# Autodesk Inventor assembly: 3 Postion Pneumatic Cylinder (9-16 in Bore, .25 in,2 in stroke)
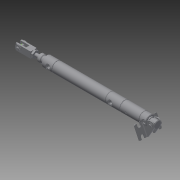
[picture p0: Inventor's stored thumbnail of the model, 180x180]
Saved by Autodesk Inventor 2014 (Build 180170000, 170)
## iProperties
Created: 2014-01-17
Part Number: 3 Postion Pneumatic Cylinder (9-16 in Bore, .25 in,2 in stroke)
Document SubType Name: Assembly
Designer: Michael
Mass: 25.114 g
Surface Area: 262.97 cm^2
Volume: 25.114 cm^3
Density: 1 g/cm^3
Title: //expscmdclustefs.cadenas.external/client_exchange/iodir/jobs/output/wkb68069816_no0/STEP/020_25_2-DXP_D-850__D-12321-A__2_03.stp
Description: STEP AP203
Sending System: PARTsolutions
Preprocessor: PSStep 15.0.47
Author: Michael
## Documents named in this file (20)
- C:\Users\Michael\Documents\GitHub\2014buildCAD\New Collector\3 Postion Pneumatic Cylinder (9-16 in Bore, .25 in,2 in stroke).iam
- C:\Users\Michael\Documents\GitHub\2014buildCAD\Imported Components\020_25_2-DXP_D-850__D-12321-A__2_03\HI_020.25_2-DXP(D-850)(D-12321-A)0_dummy.ipt
- C:\Users\Michael\Documents\GitHub\2014buildCAD\Imported Components\020_25_2-DXP_D-850__D-12321-A__2_03\HI_D-68355-XP--0.ipt
- C:\Users\Michael\Documents\GitHub\2014buildCAD\Imported Components\020_25_2-DXP_D-850__D-12321-A__2_03\HI_D-75938XP-1.188.ipt
- C:\Users\Michael\Documents\GitHub\2014buildCAD\Imported Components\020_25_2-DXP_D-850__D-12321-A__2_03\HI_D-15705rear_head.ipt
- C:\Users\Michael\Documents\GitHub\2014buildCAD\Imported Components\020_25_2-DXP_D-850__D-12321-A__2_03\HI_D-8597.ipt
- C:\Users\Michael\Documents\GitHub\2014buildCAD\Imported Components\020_25_2-DXP_D-850__D-12321-A__2_03\HI_D-12321-A-dummy.ipt
- C:\Users\Michael\Documents\GitHub\2014buildCAD\Imported Components\020_25_2-DXP_D-850__D-12321-A__2_03\HI_D-9963_pin.ipt
- C:\Users\Michael\Documents\GitHub\2014buildCAD\Imported Components\020_25_2-DXP_D-850__D-12321-A__2_03\HI_D-782_pin.ipt
- C:\Users\Michael\Documents\GitHub\2014buildCAD\Imported Components\020_25_2-DXP_D-850__D-12321-A__2_03\HI_D-9769-clevis_pin.ipt
- C:\Users\Michael\Documents\GitHub\2014buildCAD\Imported Components\020_25_2-DXP_D-850__D-12321-A__2_03\HI_D-9770-rr.ipt
- C:\Users\Michael\Documents\GitHub\2014buildCAD\Imported Components\020_25_2-DXP_D-850__D-12321-A__2_03\HI_D-7516XP-3.25.ipt
- C:\Users\Michael\Documents\GitHub\2014buildCAD\Imported Components\020_25_2-DXP_D-850__D-12321-A__2_03\HI_D-26368----0.5_rod_guide_cyl.ipt
- C:\Users\Michael\Documents\GitHub\2014buildCAD\Imported Components\020_25_2-DXP_D-850__D-12321-A__2_03\HI_D-75080.25-2XP-4.531-3pos.ipt
- C:\Users\Michael\Documents\GitHub\2014buildCAD\Imported Components\020_25_2-DXP_D-850__D-12321-A__2_03\HI_D-850-dummy.ipt
- C:\Users\Michael\Documents\GitHub\2014buildCAD\Imported Components\020_25_2-DXP_D-850__D-12321-A__2_03\HI_D-14043.ipt
- C:\Users\Michael\Documents\GitHub\2014buildCAD\Imported Components\020_25_2-DXP_D-850__D-12321-A__2_03\HI_D-12304.ipt
- C:\Users\Michael\Documents\GitHub\2014buildCAD\Imported Components\020_25_2-DXP_D-850__D-12321-A__2_03\HI_D-5406.ipt
- C:\Users\Michael\Documents\GitHub\2014buildCAD\Imported Components\020_25_2-DXP_D-850__D-12321-A__2_03\HI_D-5288.ipt
- C:\Users\Michael\Documents\GitHub\2014buildCAD\Imported Components\020_25_2-DXP_D-850__D-12321-A__2_03\HI_D-95380.25-2XP-2.106-3pos.ipt
## Components (21 placed, 21 different names)
1. NAUO1
2. NAUO2
3. NAUO3
4. NAUO4
5. NAUO5
6. NAUO6
7. NAUO7 — Mate:2, Mate:3, Flush:2
8. NAUO8 — Flush:1, Mate:1, Mate:2, Flush:2
9. NAUO9 — Flush:1, Mate:1, Mate:3
10. NAUO10
11. NAUO11
12. NAUO12
13. NAUO13
14. NAUO14
15. NAUO15
16. NAUO16
17. NAUO17
18. NAUO18
19. NAUO19
20. NAUO20
21. NAUO21
## Relationships (5: Mate 3, Flush 2)
- Flush:1 (2.2098 mm): NAUO8 ↔ NAUO9
- Mate:1: NAUO8 ↔ NAUO9
- Mate:2 (8.3998 mm): NAUO7 ↔ NAUO8
- Mate:3: NAUO7 ↔ NAUO9
- Flush:2: NAUO7 ↔ NAUO8
